# Autodesk Inventor assembly: heightSensor
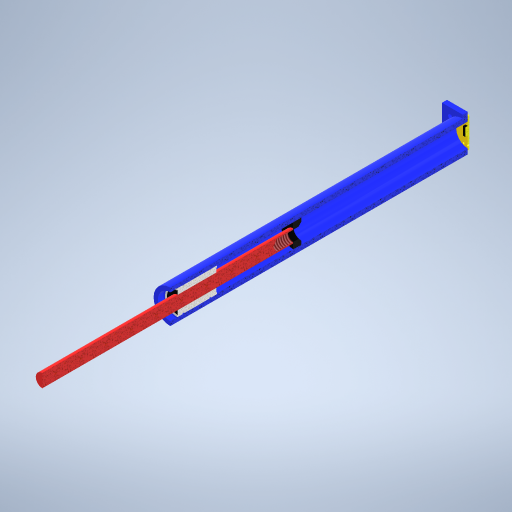
[picture p0: Inventor's stored thumbnail of the model, 512x512]
Saved by Autodesk Inventor 2023 (Build 270158000, 158)
## iProperties
Created: 2023-07-16
Part Number: heightSensor
Document SubType Name: Assembly
Designer: checo
Author: checo
## Documents named in this file (6)
- C:\Users\checo\Documents\baja_SAE_Instrumentation\CAD\height_Sensor\heightSensor.iam
- C:\Users\checo\Documents\baja_SAE_Instrumentation\CAD\height_Sensor\body.ipt
- C:\Users\checo\Documents\baja_SAE_Instrumentation\CAD\height_Sensor\plate.ipt
- C:\Users\checo\Documents\baja_SAE_Instrumentation\CAD\height_Sensor\bearing.ipt
- C:\Users\checo\Documents\baja_SAE_Instrumentation\CAD\height_Sensor\aluminium_Bar_8mm.ipt
- C:\Users\checo\Documents\baja_SAE_Instrumentation\CAD\height_Sensor\VL6180X_PCB.ipt
## Components (5 placed, 5 different names)
1. plate:1 — Mate:3, Mate:4
2. bearing:1 — Mate:1, Mate:2
3. body:1 — Mate:1, Mate:2, Mate:5, Mate:6, Mate:7, Angle:1
4. aluminium_Bar_8mm:1 — Mate:3, Mate:4, Mate:5
5. VL6180X_PCB:1 — Mate:6, Mate:7, Angle:1
## Relationships (8: Mate 7, Angle 1)
- Mate:1: bearing:1 ↔ body:1
- Mate:2: bearing:1 ↔ body:1
- Mate:3: plate:1 ↔ aluminium_Bar_8mm:1
- Mate:4: plate:1 ↔ aluminium_Bar_8mm:1
- Mate:5: body:1 ↔ aluminium_Bar_8mm:1
- Mate:6: body:1 ↔ VL6180X_PCB:1
- Mate:7: body:1 ↔ VL6180X_PCB:1
- Angle:1 (-90 deg): body:1 ↔ VL6180X_PCB:1
